# Autodesk Inventor assembly: Front Crossbrace
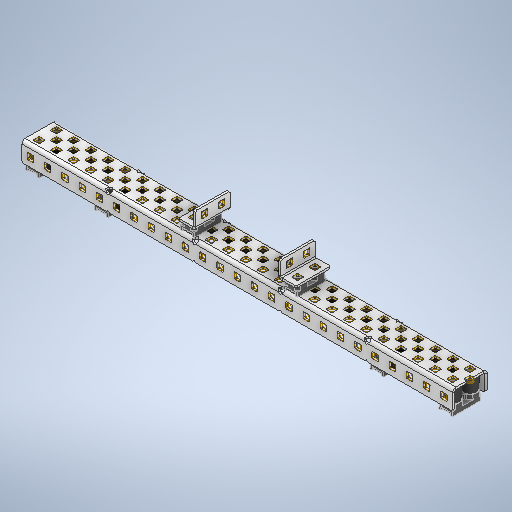
[picture p0: Inventor's stored thumbnail of the model, 512x512]
Saved by Autodesk Inventor 2025.2 (Build 292293000, 293)
## iProperties
Created: 2025-04-02
Part Number: Front Crossbrace
Document SubType Name: Assembly
Designer: avere
Author: avere
## Documents named in this file (8)
- D:\vex\cad\v5\Drivetrain\Braces\Front Crossbrace.iam
- D:\vex\cad\VEX-CAD-Inventor\Structure\C Channel\Aluminum 1x2x1\Alu C 1x2x1x25.ipt
- D:\vex\cad\VEX-CAD-Inventor\Structure\Angle\Aluminum 1x1\Alu Angle 1x1x2.ipt
- D:\vex\cad\VEX-CAD-Inventor\Motion\Shaft LS\Bearing Flat - Cut.ipt
- D:\vex\cad\VEX-CAD-Inventor\Motion\Spacers\Spacer Nylon .375 OD\NSpacer .375 OD x .375.ipt
- D:\vex\cad\VEX-CAD-Inventor\Motion\Spacers\Spacer Nylon .375 OD.ipt
- D:\vex\cad\VEX-CAD-Inventor\Motion\Spacers\Washer Steel\SWasher .375 OD x .062500.ipt
- D:\vex\cad\VEX-CAD-Inventor\Motion\Spacers\Washer Steel.ipt
## Components (25 placed, 5 different names)
1. Alu C 1x2x1x25:1 — Mate:1, Mate:2, Mate:3, Insert:1, Mate:4, Insert:2, Mate:5, Insert:3, Insert:4, Insert:9, Mate:8
2. Alu Angle 1x1x2:1 — Insert:1, Mate:4, Mate:6
3. Alu Angle 1x1x2:2 — Insert:2, Mate:5, Mate:7
4. Bearing Flat - Cut:1 — Insert:3, Mate:6
5. Bearing Flat - Cut:2 — Insert:4, Mate:7
6. Bearing Flat - Cut:4 — Insert:6, Insert:8, Mate:8
7. NSpacer .375 OD x .375:1 — Insert:5, Insert:6
8. SWasher .375 OD x .062500:1 — Insert:5, Insert:9
9. NSpacer .375 OD x .375:2 — Insert:8
10. SWasher .375 OD x .062500:2
11. Bearing Flat - Cut:5
12. NSpacer .375 OD x .375:3
13. SWasher .375 OD x .062500:3
14. NSpacer .375 OD x .375:4
15. SWasher .375 OD x .062500:4
16. Bearing Flat - Cut:6
17. NSpacer .375 OD x .375:5
18. SWasher .375 OD x .062500:5
19. NSpacer .375 OD x .375:6
20. SWasher .375 OD x .062500:6
21. Bearing Flat - Cut:7
22. NSpacer .375 OD x .375:7
23. SWasher .375 OD x .062500:7
24. NSpacer .375 OD x .375:8
25. SWasher .375 OD x .062500:8
## Component patterns: (4 elements, first: Bearing Flat - Cut:4 + NSpacer .375 OD x .375:1 + SWasher .375 OD x .062500:1 + NSpacer .375 OD x .375:2 + SWasher .375 OD x .062500:2)
## Relationships (17: Insert 9, Mate 8)
- Mate:1 (25.4 mm): Alu C 1x2x1x25:1
- Mate:2 (-158.75 mm): Alu C 1x2x1x25:1
- Mate:3 (50.8 mm): Alu C 1x2x1x25:1
- Insert:1 (6.35 mm): Alu C 1x2x1x25:1 ↔ Alu Angle 1x1x2:1
- Mate:4: Alu C 1x2x1x25:1 ↔ Alu Angle 1x1x2:1
- Insert:2 (6.35 mm): Alu C 1x2x1x25:1 ↔ Alu Angle 1x1x2:2
- Mate:5: Alu C 1x2x1x25:1 ↔ Alu Angle 1x1x2:2
- Insert:3: Alu C 1x2x1x25:1 ↔ Bearing Flat - Cut:1
- Mate:6: Alu Angle 1x1x2:1 ↔ Bearing Flat - Cut:1
- Insert:4: Alu C 1x2x1x25:1 ↔ Bearing Flat - Cut:2
- Mate:7: Alu Angle 1x1x2:2 ↔ Bearing Flat - Cut:2
- Insert:5: NSpacer .375 OD x .375:1 ↔ SWasher .375 OD x .062500:1
- Insert:6: Bearing Flat - Cut:4 ↔ NSpacer .375 OD x .375:1
- [Insert]: NSpacer .375 OD x .375:2 ↔ SWasher .375 OD x .062500:2
- Insert:8: Bearing Flat - Cut:4 ↔ NSpacer .375 OD x .375:2
- Insert:9: Alu C 1x2x1x25:1 ↔ SWasher .375 OD x .062500:1
- Mate:8: Alu C 1x2x1x25:1 ↔ Bearing Flat - Cut:4
## Named parameters: d13_d11 = 0 mm
